# Autodesk Inventor assembly: Synchronous Belts Transmission3_MIR1
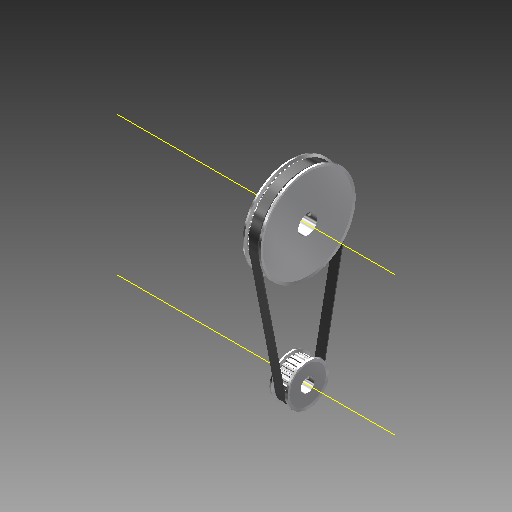
[picture p0: Inventor's stored thumbnail of the model, 512x512]
Saved by Autodesk Inventor 2019 (Build 230136000, 136)
## iProperties
Created: 2019-10-19
Part Number: Synchronous Belts Transmission3_MIR1
Document SubType Name: Assembly
Designer: admin
Author: admin
## Documents named in this file (4)
- C:\Users\Mark\Desktop\7738 Helion Engineering\7738-CAD-prep\Butterfly drive\Butterfly Drive Module\Design Accelerator\Synchronous Belts Transmission3_MIR1.iam
- C:\Users\Mark\Desktop\7738 Helion Engineering\7738-CAD-prep\Butterfly drive\Butterfly Drive Module\Design Accelerator\Synchronous Belt3_MIR1.ipt
- C:\Users\Mark\Desktop\7738 Helion Engineering\7738-CAD-prep\Butterfly drive\Butterfly Drive Module\Design Accelerator\Synchronous Pulley13_MIR1.ipt
- C:\Users\Mark\Desktop\7738 Helion Engineering\7738-CAD-prep\Butterfly drive\Butterfly Drive Module\Design Accelerator\Synchronous Pulley23_MIR1.ipt
## Components (3 placed, 3 different names)
1. Synchronous Belt3_MIR1:1 — Mate:2, Mate:1, Flush:1, Mate:4, Mate:3, Flush:2
2. Synchronous Pulley13_MIR1:1 — Mate:2, Mate:1, Flush:1, Rotation:1
3. Synchronous Pulley23_MIR1:1 — Mate:4, Mate:3, Flush:2, Rotation:1
## Relationships (7: Flush 4, Mate 2, RelateRotation 1)
- Mate:2 [Flush]: Synchronous Belt3_MIR1:1 ↔ Synchronous Pulley13_MIR1:1
- Mate:1: Synchronous Belt3_MIR1:1 ↔ Synchronous Pulley13_MIR1:1
- Flush:1: Synchronous Belt3_MIR1:1 ↔ Synchronous Pulley13_MIR1:1
- Mate:4 [Flush]: Synchronous Belt3_MIR1:1 ↔ Synchronous Pulley23_MIR1:1
- Mate:3: Synchronous Belt3_MIR1:1 ↔ Synchronous Pulley23_MIR1:1
- Flush:2: Synchronous Belt3_MIR1:1 ↔ Synchronous Pulley23_MIR1:1
- Rotation:1 [RelateRotation] (2.4 ul): Synchronous Pulley13_MIR1:1 ↔ Synchronous Pulley23_MIR1:1
